# Autodesk Inventor assembly: 02하체
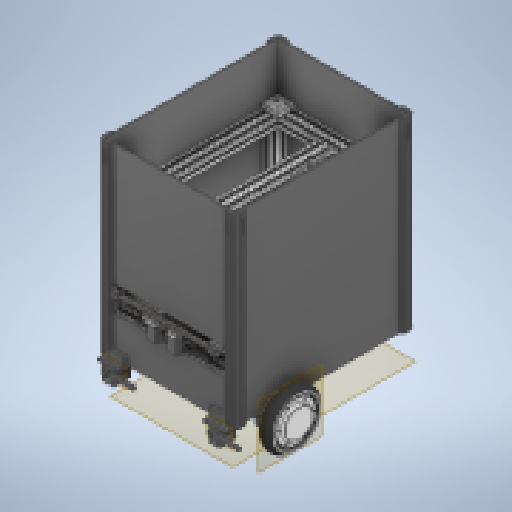
[picture p0: Inventor's stored thumbnail of the model, 512x512]
Saved by Autodesk Inventor 2026.2 (Build 302298010, 298A)
## iProperties
Created: 2026-03-27
Part Number: 02하체
Document SubType Name: Assembly
Designer: chanh
Author: chanh
## Documents named in this file (48)
- C:\Users\chanh\내 드라이브\교과공부\2026년 1학기 (4학년 1학기)\01창의제품설계\UMMA_CAD\02하체\02하체.iam
- C:\Users\chanh\내 드라이브\교과공부\2026년 1학기 (4학년 1학기)\01창의제품설계\UMMA_CAD\02하체\3060 Aluminium Profile 450mm.ipt
- C:\Users\chanh\내 드라이브\교과공부\2026년 1학기 (4학년 1학기)\01창의제품설계\UMMA_CAD\02하체\3060 Aluminium Profile 480mm.ipt
- C:\Users\chanh\내 드라이브\교과공부\2026년 1학기 (4학년 1학기)\01창의제품설계\UMMA_CAD\00부품\ZLLG80ASM250-L V3.0 (모터)\ZLLG80ASM250-L V3.0 Single shaft.iam
- C:\Users\chanh\내 드라이브\교과공부\2026년 1학기 (4학년 1학기)\01창의제품설계\UMMA_CAD\00부품\ZLAC8015D V4.0 (드라이버)\ZLAC8015D V4.0.iam
- C:\Users\chanh\내 드라이브\교과공부\2026년 1학기 (4학년 1학기)\01창의제품설계\UMMA_CAD\00부품\ZLLG80ASM250-L V3.0 (모터)\Nut.ipt
- C:\Users\chanh\내 드라이브\교과공부\2026년 1학기 (4학년 1학기)\01창의제품설계\UMMA_CAD\02하체\motor_bracket.ipt
- C:\Users\chanh\내 드라이브\교과공부\2026년 1학기 (4학년 1학기)\01창의제품설계\UMMA_CAD\02하체\Bottom_Plate_Acryl.ipt
- C:\Users\chanh\내 드라이브\교과공부\2026년 1학기 (4학년 1학기)\01창의제품설계\UMMA_CAD\02하체\Battery.ipt
- C:\Users\chanh\내 드라이브\교과공부\2026년 1학기 (4학년 1학기)\01창의제품설계\UMMA_CAD\02하체\assist_wheel.iam
- C:\Users\chanh\내 드라이브\교과공부\2026년 1학기 (4학년 1학기)\01창의제품설계\UMMA_CAD\02하체\assist_wheel_bracket.ipt
- C:\Users\chanh\내 드라이브\교과공부\2026년 1학기 (4학년 1학기)\01창의제품설계\UMMA_CAD\02하체\3060 Aluminium Profile 410mm.ipt
- C:\Users\chanh\내 드라이브\교과공부\2026년 1학기 (4학년 1학기)\01창의제품설계\UMMA_CAD\02하체\3060 Aluminium Profile 390mm.ipt
- C:\Users\chanh\내 드라이브\교과공부\2026년 1학기 (4학년 1학기)\01창의제품설계\UMMA_CAD\02하체\Linear Motor Bar (T-Frame).ipt
- C:\Users\chanh\내 드라이브\교과공부\2026년 1학기 (4학년 1학기)\01창의제품설계\UMMA_CAD\02하체\Linear Motor (T-Frame).ipt
- C:\Users\chanh\내 드라이브\교과공부\2026년 1학기 (4학년 1학기)\01창의제품설계\UMMA_CAD\02하체\Linear Motor Rear Braket.ipt
- C:\Users\chanh\내 드라이브\교과공부\2026년 1학기 (4학년 1학기)\01창의제품설계\UMMA_CAD\02하체\Linear Motor Front Braket.ipt
- C:\Users\chanh\내 드라이브\교과공부\2026년 1학기 (4학년 1학기)\01창의제품설계\UMMA_CAD\02하체\LMF20UU.ipt
- C:\Users\chanh\내 드라이브\교과공부\2026년 1학기 (4학년 1학기)\01창의제품설계\UMMA_CAD\02하체\Lift Bracket other side.ipt
- C:\Users\chanh\내 드라이브\교과공부\2026년 1학기 (4학년 1학기)\01창의제품설계\UMMA_CAD\02하체\Lift Bracket.ipt
- C:\Users\chanh\내 드라이브\교과공부\2026년 1학기 (4학년 1학기)\01창의제품설계\UMMA_CAD\02하체\MGN15C Cart.ipt
- C:\Users\chanh\내 드라이브\교과공부\2026년 1학기 (4학년 1학기)\01창의제품설계\UMMA_CAD\02하체\MGN15 Rail.ipt
- C:\Users\chanh\내 드라이브\교과공부\2026년 1학기 (4학년 1학기)\01창의제품설계\UMMA_CAD\02하체\Linear Motor Mount Right.ipt
- C:\Users\chanh\내 드라이브\교과공부\2026년 1학기 (4학년 1학기)\01창의제품설계\UMMA_CAD\02하체\Linear Motor Mount Left.ipt
- C:\Users\chanh\내 드라이브\교과공부\2026년 1학기 (4학년 1학기)\01창의제품설계\UMMA_CAD\02하체\LM Cart Braket.ipt
- C:\Users\chanh\내 드라이브\교과공부\2026년 1학기 (4학년 1학기)\01창의제품설계\UMMA_CAD\02하체\Space Craft Braket.ipt
- C:\Users\chanh\내 드라이브\교과공부\2026년 1학기 (4학년 1학기)\01창의제품설계\UMMA_CAD\02하체\LM20UU.ipt
- C:\Users\chanh\내 드라이브\교과공부\2026년 1학기 (4학년 1학기)\01창의제품설계\UMMA_CAD\02하체\Power Box (12V).ipt
- C:\Users\chanh\내 드라이브\교과공부\2026년 1학기 (4학년 1학기)\01창의제품설계\UMMA_CAD\02하체\Power Box (24V).ipt
- C:\Users\chanh\내 드라이브\교과공부\2026년 1학기 (4학년 1학기)\01창의제품설계\UMMA_CAD\02하체\Limit SW Bracket Right.ipt
- C:\Users\chanh\내 드라이브\교과공부\2026년 1학기 (4학년 1학기)\01창의제품설계\UMMA_CAD\02하체\Limit SW Bracket Left.ipt
- C:\Users\chanh\내 드라이브\교과공부\2026년 1학기 (4학년 1학기)\01창의제품설계\UMMA_CAD\02하체\RE38S-600Z-1M.ipt
- C:\Users\chanh\내 드라이브\교과공부\2026년 1학기 (4학년 1학기)\01창의제품설계\UMMA_CAD\02하체\Lift_encoder_frame.ipt
- C:\Users\chanh\내 드라이브\교과공부\2026년 1학기 (4학년 1학기)\01창의제품설계\UMMA_CAD\02하체\RE38S-600Z-1M-no-end.ipt
- C:\Users\chanh\내 드라이브\교과공부\2026년 1학기 (4학년 1학기)\01창의제품설계\UMMA_CAD\02하체\T-Frame_encoder_frame.ipt
- C:\Users\chanh\내 드라이브\교과공부\2026년 1학기 (4학년 1학기)\01창의제품설계\UMMA_CAD\02하체\LED Power Box (12V).ipt
- C:\Users\chanh\내 드라이브\교과공부\2026년 1학기 (4학년 1학기)\01창의제품설계\UMMA_CAD\02하체\LED Power Box (12V) Pillar.ipt
- C:\Users\chanh\내 드라이브\교과공부\2026년 1학기 (4학년 1학기)\01창의제품설계\UMMA_CAD\02하체\LED Power Box (12V) Cover.ipt
- C:\Users\chanh\내 드라이브\교과공부\2026년 1학기 (4학년 1학기)\01창의제품설계\UMMA_CAD\02하체\Power Box (24V) Cover.ipt
- C:\Users\chanh\내 드라이브\교과공부\2026년 1학기 (4학년 1학기)\01창의제품설계\UMMA_CAD\02하체\Power Box (12V) Cover.ipt
- C:\Users\chanh\내 드라이브\교과공부\2026년 1학기 (4학년 1학기)\01창의제품설계\UMMA_CAD\02하체\MGN15 Rail Middle.ipt
- C:\Users\chanh\내 드라이브\교과공부\2026년 1학기 (4학년 1학기)\01창의제품설계\UMMA_CAD\02하체\T-Frame Left Cover.ipt
- C:\Users\chanh\내 드라이브\교과공부\2026년 1학기 (4학년 1학기)\01창의제품설계\UMMA_CAD\02하체\T-Frame Right Cover.ipt
- C:\Users\chanh\내 드라이브\교과공부\2026년 1학기 (4학년 1학기)\01창의제품설계\UMMA_CAD\02하체\Foam Sheet Side.ipt
- C:\Users\chanh\내 드라이브\교과공부\2026년 1학기 (4학년 1학기)\01창의제품설계\UMMA_CAD\02하체\Foam Sheet Front.ipt
- C:\Users\chanh\내 드라이브\교과공부\2026년 1학기 (4학년 1학기)\01창의제품설계\UMMA_CAD\02하체\Foam Sheet Back.ipt
- C:\Users\chanh\내 드라이브\교과공부\2026년 1학기 (4학년 1학기)\01창의제품설계\UMMA_CAD\02하체\Foam Sheet Corner.ipt
- C:\Users\chanh\내 드라이브\교과공부\2026년 1학기 (4학년 1학기)\01창의제품설계\UMMA_CAD\02하체\Stopper\stopper.iam
## Components (79 placed, 47 different names)
1. stopper:1 [sub-assembly] — Mate:113, Flush:90, Mate:114
2. Lift Bracket:2 — Flush:59, Flush:60, Mate:40
3. Lift Bracket:1 — Flush:57, Mate:39, Flush:58
4. Lift Bracket other side:2 — Mate:42, Flush:63, Flush:64
5. Lift Bracket other side:1 — Mate:41, Flush:61, Flush:62
6. 3060 Aluminium Profile 480mm:1 — Mate:2, Flush:6, Flush:7, Mate:4, Flush:8, Flush:9, Flush:10, Flush:17, Mate:15, Mate:107, Flush:84
7. 3060 Aluminium Profile 480mm:2 — Mate:3, Flush:4, Flush:5, Flush:11, Mate:13, Mate:14, Mate:108, Flush:86
8. 3060 Aluminium Profile 480mm:3 — Flush:13, Mate:8, Flush:14, Mate:9
9. 3060 Aluminium Profile 480mm:4 — Flush:31, Mate:25, Flush:38
10. 3060 Aluminium Profile 480mm:5 — Flush:30, Mate:24, Flush:37
11. 3060 Aluminium Profile 480mm:6 — Flush:32, Mate:26, Flush:39, Flush:79, Mate:86, Mate:88, Flush:81
12. 3060 Aluminium Profile 480mm:7 — Mate:30, Flush:43, Flush:44, Mate:31, Flush:45, Mate:35, Flush:47, Mate:89, Mate:90, Mate:91, Mate:92, Mate:99
13. 3060 Aluminium Profile 450mm:1 — Flush:2, Mate:1, Flush:3, Mate:2, Mate:3, Flush:4, Flush:5, Flush:6, Flush:7, Mate:18, Mate:21, Flush:24, Flush:25, Flush:26, Flush:27, Flush:88, Flush:90, Mate:114
14. 3060 Aluminium Profile 450mm:2 — Mate:4, Flush:8, Flush:9, Flush:13, Mate:8, Mate:16, Flush:18, Mate:20, Flush:22, Flush:23, Mate:19, Flush:28, Flush:29, Mate:28
15. 3060 Aluminium Profile 450mm:3 — Mate:22, Flush:35, Flush:36, Mate:24, Flush:37, Mate:25, Flush:38, Mate:26, Flush:57, Mate:39, Flush:58, Mate:42, Flush:63, Flush:64, Mate:87
16. 3060 Aluminium Profile 450mm:4 — Mate:23, Flush:30, Flush:31, Flush:32, Flush:33, Flush:34, Flush:39, Flush:59, Flush:60, Mate:40, Mate:41, Flush:61, Flush:62
17. 3060 Aluminium Profile 410mm:1 — Mate:19, Flush:28, Flush:29, Mate:22, Mate:27, Flush:40
18. 3060 Aluminium Profile 410mm:2 — Mate:18, Flush:26, Flush:27, Mate:23, Mate:29, Flush:41, Mate:85, Flush:85
19. 3060 Aluminium Profile 410mm:3 — Mate:21, Flush:24, Flush:25, Flush:33, Flush:34, Mate:83, Flush:87
20. 3060 Aluminium Profile 410mm:4 — Mate:20, Flush:22, Flush:23, Flush:35, Flush:36
21. 3060 Aluminium Profile 390mm:1 — Mate:29, Flush:41, Flush:42, Flush:43, Flush:55, Mate:38, Flush:77, Mate:82, Mate:84, Flush:78, Mate:109
22. 3060 Aluminium Profile 390mm:2 — Mate:27, Flush:40, Mate:28, Flush:42, Mate:30, Flush:44, Flush:49, Flush:50, Mate:37, Mate:111
23. T-Frame Left Cover:1 — Rigid:21
24. T-Frame Right Cover:1 — Rigid:22
25. MGN15 Rail Middle:1 — Mate:106, Rotational:1
26. MGN15C Cart:4 — Rigid:20
27. MGN15C Cart:1 — Slider:2, Rigid:8
28. MGN15 Rail:1 — Slider:1, Slider:2, Rigid:21, Rigid:22, Rotational:1
29. MGN15C Cart:2 — Slider:1, Flush:67, Flush:68, Mate:67
30. Linear Motor Mount Right:1 — Rigid:7, Mate:72
31. Linear Motor Mount Left:1 — Rigid:9, Mate:73, Mate:105
32. LM Cart Braket:1 — Flush:67, Flush:68, Mate:67, Mate:72
33. LM Cart Braket:2 — Rigid:8, Mate:73, Mate:105
34. Space Craft Braket:1 — Rigid:10, Rigid:11, Mate:104, Rigid:20
35. LM20UU:1 — Rigid:10, Mate:69
36. LM20UU:2 — Rigid:11, Mate:68
37. Linear Motor Front Braket:1 — Flush:55, Flush:56, Mate:38, Rigid:5, Rigid:6, Mate:93, Mate:97, Angle:4, Mate:98, Angle:5
38. LMF20UU:1 — Rigid:5, Mate:104
39. LMF20UU:2 — Rigid:6
40. Linear Motor (T-Frame):1 — Mate:31, Flush:45, Mate:32, Angle:2, T자 왼쪽 거리, Flush:53
41. Linear Motor Bar (T-Frame):1 — Mate:32, Angle:2, T자 왼쪽 거리, Rigid:7, Mate:69
42. Linear Motor (T-Frame):2 — T자 오른쪽 거리, Mate:34, Angle:3, Mate:35, Flush:47, Flush:54
43. Linear Motor Bar (T-Frame):2 — T자 오른쪽 거리, Mate:34, Angle:3, Rigid:9, Mate:68
44. Linear Motor Rear Braket:1 — Flush:49, Flush:50, Mate:37, Flush:53, Flush:54, Mate:100, Mate:101
45. ZLLG80ASM250-L V3.0 Single shaft:1 [sub-assembly] — Rigid:3
46. ZLLG80ASM250-L V3.0 Single shaft:2 [sub-assembly] — Rigid:1
47. Nut:1 — Rigid:2
48. Nut:2 — Rigid:4
49. motor_bracket:1 — Flush:10, Flush:17, Rigid:1, Rigid:2, Mate:15
50. motor_bracket:2 — Flush:11, Mate:13, Rigid:3, Rigid:4, Mate:14
51. assist_wheel:1 [sub-assembly] — Tangent:1, Mate:17, Flush:20, Flush:21
52. assist_wheel_bracket:1 — Mate:16, Flush:18, Flush:19, Mate:17, Flush:20
53. Power Box (24V) Cover:1 — Rigid:18
54. Power Box (12V) Cover:1 — Rigid:19
55. ZLAC8015D V4.0:2 [sub-assembly] — Mate:102, Mate:103, Flush:83
56. LED Power Box (12V):1 — Rigid:15, Rigid:16, Rigid:17
57. LED Power Box (12V) Pillar:1 — Rigid:15
58. LED Power Box (12V) Pillar:2 — Rigid:16, Mate:99, Mate:100, Mate:101
59. LED Power Box (12V) Cover:1 — Rigid:17
60. Limit SW Bracket Right:1 — Flush:77, Mate:82, Mate:83
61. Limit SW Bracket Left:1 — Mate:84, Flush:78, Mate:85
62. Power Box (24V):1 — Mate:79, Mate:80, Mate:81, Rigid:18
63. Power Box (12V):1 — Mate:75, Flush:76, Mate:78, Mate:80, Rigid:19
64. Battery:1 — Mate:11, Flush:73, Flush:74, Mate:103, Flush:83
65. Bottom_Plate_Acryl:1 — Mate:9, Flush:15, Flush:16, Mate:11, Angle:1, Flush:74, Mate:75, Flush:76, Mate:79, Mate:102
66. RE38S-600Z-1M:1 — Flush:79, Mate:86, Mate:87, Flush:80
67. Lift_encoder_frame:1 — Flush:80, Mate:88, Flush:81
68. RE38S-600Z-1M-no-end:1 — Mate:92, Mate:89, Flush:82, Mate:93, Mate:94, Mate:95, Mate:96
69. RE38S-600Z-1M-no-end:2 — Mate:91, Mate:90, Flush:82, Rigid:14
70. T-Frame_encoder_frame:1 — Mate:94, Mate:95, Mate:96
71. T-Frame_encoder_frame:2 — Rigid:14
72. Foam Sheet Side:1 — Mate:107, Flush:84, Flush:85, Flush:89, Mate:112, Rigid:24
73. Foam Sheet Side:2 — Mate:108, Flush:86, Flush:87, Mate:110, Rigid:23, Rigid:26
74. Foam Sheet Front:1 — Mate:109, Flush:88, Mate:110, Mate:113
75. Foam Sheet Back:1 — Mate:111, Flush:89, Mate:112, Rigid:25
76. Foam Sheet Corner:1 — Rigid:23
77. Foam Sheet Corner:2 — Rigid:25
78. Foam Sheet Corner:3 — Rigid:26
79. Foam Sheet Corner:4 — Rigid:24
## Relationships (191: Mate 80, Flush 78, WeldJoint 24, Angle 5, TranslationJoint 2, Tangent 1, RevoluteJoint 1)
- T자 왼쪽 거리 [Mate] (87 mm): Linear Motor (T-Frame):1 ↔ Linear Motor Bar (T-Frame):1
- T자 오른쪽 거리 [Mate] (87 mm): Linear Motor (T-Frame):2 ↔ Linear Motor Bar (T-Frame):2
- Flush:1 (-240 mm)
- Flush:2: 3060 Aluminium Profile 450mm:1
- Mate:1: 3060 Aluminium Profile 450mm:1
- Flush:3: 3060 Aluminium Profile 450mm:1
- Mate:2: 3060 Aluminium Profile 480mm:1 ↔ 3060 Aluminium Profile 450mm:1
- Mate:3: 3060 Aluminium Profile 480mm:2 ↔ 3060 Aluminium Profile 450mm:1
- Flush:4: 3060 Aluminium Profile 480mm:2 ↔ 3060 Aluminium Profile 450mm:1
- Flush:5: 3060 Aluminium Profile 480mm:2 ↔ 3060 Aluminium Profile 450mm:1
- Flush:6: 3060 Aluminium Profile 480mm:1 ↔ 3060 Aluminium Profile 450mm:1
- Flush:7: 3060 Aluminium Profile 480mm:1 ↔ 3060 Aluminium Profile 450mm:1
- Mate:4: 3060 Aluminium Profile 480mm:1 ↔ 3060 Aluminium Profile 450mm:2
- Flush:8: 3060 Aluminium Profile 480mm:1 ↔ 3060 Aluminium Profile 450mm:2
- Flush:9: 3060 Aluminium Profile 480mm:1 ↔ 3060 Aluminium Profile 450mm:2
- Flush:10: 3060 Aluminium Profile 480mm:1 ↔ motor_bracket:1
- Flush:17 (150 mm): 3060 Aluminium Profile 480mm:1 ↔ motor_bracket:1
- Rigid:1 [WeldJoint]: ZLLG80ASM250-L V3.0 Single shaft:2 ↔ motor_bracket:1
- Rigid:2 [WeldJoint]: Nut:1 ↔ motor_bracket:1
- Flush:11: 3060 Aluminium Profile 480mm:2 ↔ motor_bracket:2
- Mate:13 (-150 mm): 3060 Aluminium Profile 480mm:2 ↔ motor_bracket:2
- Rigid:3 [WeldJoint]: ZLLG80ASM250-L V3.0 Single shaft:1 ↔ motor_bracket:2
- Rigid:4 [WeldJoint]: Nut:2 ↔ motor_bracket:2
- Flush:13: 3060 Aluminium Profile 480mm:3 ↔ 3060 Aluminium Profile 450mm:2
- Mate:8: 3060 Aluminium Profile 480mm:3 ↔ 3060 Aluminium Profile 450mm:2
- Flush:14: 3060 Aluminium Profile 480mm:3
- Mate:9: 3060 Aluminium Profile 480mm:3 ↔ Bottom_Plate_Acryl:1
- Flush:15: Bottom_Plate_Acryl:1
- Flush:16: Bottom_Plate_Acryl:1
- Mate:11: Battery:1 ↔ Bottom_Plate_Acryl:1
- Mate:14: 3060 Aluminium Profile 480mm:2 ↔ motor_bracket:2
- Mate:15: 3060 Aluminium Profile 480mm:1 ↔ motor_bracket:1
- Angle:1 (0 deg): Bottom_Plate_Acryl:1
- Tangent:1: assist_wheel:1
- Mate:16: 3060 Aluminium Profile 450mm:2 ↔ assist_wheel_bracket:1
- Flush:18: 3060 Aluminium Profile 450mm:2 ↔ assist_wheel_bracket:1
- Flush:19: assist_wheel_bracket:1
- Mate:17: assist_wheel:1 ↔ assist_wheel_bracket:1
- Flush:20: assist_wheel:1 ↔ assist_wheel_bracket:1
- Flush:21: assist_wheel:1
- Mate:18: 3060 Aluminium Profile 450mm:1 ↔ 3060 Aluminium Profile 410mm:2
- Mate:19: 3060 Aluminium Profile 450mm:2 ↔ 3060 Aluminium Profile 410mm:1
- Mate:20: 3060 Aluminium Profile 450mm:2 ↔ 3060 Aluminium Profile 410mm:4
- Mate:21: 3060 Aluminium Profile 450mm:1 ↔ 3060 Aluminium Profile 410mm:3
- Flush:22: 3060 Aluminium Profile 450mm:2 ↔ 3060 Aluminium Profile 410mm:4
- Flush:23: 3060 Aluminium Profile 450mm:2 ↔ 3060 Aluminium Profile 410mm:4
- Flush:24: 3060 Aluminium Profile 450mm:1 ↔ 3060 Aluminium Profile 410mm:3
- Flush:25: 3060 Aluminium Profile 450mm:1 ↔ 3060 Aluminium Profile 410mm:3
- Flush:26: 3060 Aluminium Profile 450mm:1 ↔ 3060 Aluminium Profile 410mm:2
- Flush:27: 3060 Aluminium Profile 450mm:1 ↔ 3060 Aluminium Profile 410mm:2
- Flush:28: 3060 Aluminium Profile 450mm:2 ↔ 3060 Aluminium Profile 410mm:1
- Flush:29: 3060 Aluminium Profile 450mm:2 ↔ 3060 Aluminium Profile 410mm:1
- Mate:22: 3060 Aluminium Profile 450mm:3 ↔ 3060 Aluminium Profile 410mm:1
- Mate:23: 3060 Aluminium Profile 450mm:4 ↔ 3060 Aluminium Profile 410mm:2
- Flush:30: 3060 Aluminium Profile 480mm:5 ↔ 3060 Aluminium Profile 450mm:4
- Flush:31: 3060 Aluminium Profile 480mm:4 ↔ 3060 Aluminium Profile 450mm:4
- Flush:32: 3060 Aluminium Profile 480mm:6 ↔ 3060 Aluminium Profile 450mm:4
- Flush:33: 3060 Aluminium Profile 450mm:4 ↔ 3060 Aluminium Profile 410mm:3
- Flush:34: 3060 Aluminium Profile 450mm:4 ↔ 3060 Aluminium Profile 410mm:3
- Flush:35: 3060 Aluminium Profile 450mm:3 ↔ 3060 Aluminium Profile 410mm:4
- Flush:36: 3060 Aluminium Profile 450mm:3 ↔ 3060 Aluminium Profile 410mm:4
- Mate:24: 3060 Aluminium Profile 480mm:5 ↔ 3060 Aluminium Profile 450mm:3
- Flush:37: 3060 Aluminium Profile 480mm:5 ↔ 3060 Aluminium Profile 450mm:3
- Mate:25: 3060 Aluminium Profile 480mm:4 ↔ 3060 Aluminium Profile 450mm:3
- Flush:38: 3060 Aluminium Profile 480mm:4 ↔ 3060 Aluminium Profile 450mm:3
- Mate:26: 3060 Aluminium Profile 480mm:6 ↔ 3060 Aluminium Profile 450mm:3
- Flush:39: 3060 Aluminium Profile 480mm:6 ↔ 3060 Aluminium Profile 450mm:4
- Mate:27: 3060 Aluminium Profile 410mm:1 ↔ 3060 Aluminium Profile 390mm:2
- Flush:40: 3060 Aluminium Profile 410mm:1 ↔ 3060 Aluminium Profile 390mm:2
- Mate:28 (80 mm): 3060 Aluminium Profile 450mm:2 ↔ 3060 Aluminium Profile 390mm:2
- Mate:29: 3060 Aluminium Profile 410mm:2 ↔ 3060 Aluminium Profile 390mm:1
- Flush:41: 3060 Aluminium Profile 410mm:2 ↔ 3060 Aluminium Profile 390mm:1
- Flush:42: 3060 Aluminium Profile 390mm:1 ↔ 3060 Aluminium Profile 390mm:2
- Mate:30: 3060 Aluminium Profile 480mm:7 ↔ 3060 Aluminium Profile 390mm:2
- Flush:43: 3060 Aluminium Profile 480mm:7 ↔ 3060 Aluminium Profile 390mm:1
- Flush:44: 3060 Aluminium Profile 480mm:7 ↔ 3060 Aluminium Profile 390mm:2
- Mate:31 (10 mm): 3060 Aluminium Profile 480mm:7 ↔ Linear Motor (T-Frame):1
- Flush:45 (-35 mm): 3060 Aluminium Profile 480mm:7 ↔ Linear Motor (T-Frame):1
- Mate:32: Linear Motor (T-Frame):1 ↔ Linear Motor Bar (T-Frame):1
- Angle:2 (-20 deg): Linear Motor (T-Frame):1 ↔ Linear Motor Bar (T-Frame):1
- Mate:34: Linear Motor (T-Frame):2 ↔ Linear Motor Bar (T-Frame):2
- Angle:3 (20 deg): Linear Motor (T-Frame):2 ↔ Linear Motor Bar (T-Frame):2
- Mate:35 (10 mm): 3060 Aluminium Profile 480mm:7 ↔ Linear Motor (T-Frame):2
- Flush:47 (-35 mm): 3060 Aluminium Profile 480mm:7 ↔ Linear Motor (T-Frame):2
- Flush:49: 3060 Aluminium Profile 390mm:2 ↔ Linear Motor Rear Braket:1
- Flush:50: 3060 Aluminium Profile 390mm:2 ↔ Linear Motor Rear Braket:1
- Mate:37: 3060 Aluminium Profile 390mm:2 ↔ Linear Motor Rear Braket:1
- Flush:53 (15 mm): Linear Motor (T-Frame):1 ↔ Linear Motor Rear Braket:1
- Flush:54 (15 mm): Linear Motor (T-Frame):2 ↔ Linear Motor Rear Braket:1
- Flush:55 (60 mm): 3060 Aluminium Profile 390mm:1 ↔ Linear Motor Front Braket:1
- Flush:56: Linear Motor Front Braket:1
- Mate:38: 3060 Aluminium Profile 390mm:1 ↔ Linear Motor Front Braket:1
- Rigid:5 [WeldJoint]: Linear Motor Front Braket:1 ↔ LMF20UU:1
- Rigid:6 [WeldJoint]: Linear Motor Front Braket:1 ↔ LMF20UU:2
- Flush:57: Lift Bracket:1 ↔ 3060 Aluminium Profile 450mm:3
- Mate:39: Lift Bracket:1 ↔ 3060 Aluminium Profile 450mm:3
- Flush:58 (1 mm): Lift Bracket:1 ↔ 3060 Aluminium Profile 450mm:3
- Flush:59: Lift Bracket:2 ↔ 3060 Aluminium Profile 450mm:4
- Flush:60 (1 mm): Lift Bracket:2 ↔ 3060 Aluminium Profile 450mm:4
- Mate:40: Lift Bracket:2 ↔ 3060 Aluminium Profile 450mm:4
- Mate:41: Lift Bracket other side:1 ↔ 3060 Aluminium Profile 450mm:4
- Flush:61 (1 mm): Lift Bracket other side:1 ↔ 3060 Aluminium Profile 450mm:4
- Flush:62: Lift Bracket other side:1 ↔ 3060 Aluminium Profile 450mm:4
- Mate:42: Lift Bracket other side:2 ↔ 3060 Aluminium Profile 450mm:3
- Flush:63: Lift Bracket other side:2 ↔ 3060 Aluminium Profile 450mm:3
- Flush:64 (1 mm): Lift Bracket other side:2 ↔ 3060 Aluminium Profile 450mm:3
- Slider:1 [TranslationJoint]: MGN15 Rail:1 ↔ MGN15C Cart:2
- Slider:2 [TranslationJoint]: MGN15C Cart:1 ↔ MGN15 Rail:1
- Rigid:7 [WeldJoint]: Linear Motor Mount Right:1 ↔ Linear Motor Bar (T-Frame):1
- Flush:67: MGN15C Cart:2 ↔ LM Cart Braket:1
- Flush:68: MGN15C Cart:2 ↔ LM Cart Braket:1
- Mate:67: MGN15C Cart:2 ↔ LM Cart Braket:1
- Rigid:8 [WeldJoint]: MGN15C Cart:1 ↔ LM Cart Braket:2
- Rigid:9 [WeldJoint]: Linear Motor Mount Left:1 ↔ Linear Motor Bar (T-Frame):2
- Rigid:10 [WeldJoint]: Space Craft Braket:1 ↔ LM20UU:1
- Rigid:11 [WeldJoint]: Space Craft Braket:1 ↔ LM20UU:2
- Mate:68: LM20UU:2 ↔ Linear Motor Bar (T-Frame):2
- Mate:69: LM20UU:1 ↔ Linear Motor Bar (T-Frame):1
- Mate:72: Linear Motor Mount Right:1 ↔ LM Cart Braket:1
- Mate:73: Linear Motor Mount Left:1 ↔ LM Cart Braket:2
- Flush:73: Battery:1
- Flush:74: Battery:1 ↔ Bottom_Plate_Acryl:1
- Mate:75: Power Box (12V):1 ↔ Bottom_Plate_Acryl:1
- Flush:76: Power Box (12V):1 ↔ Bottom_Plate_Acryl:1
- Mate:78: Power Box (12V):1
- Mate:79: Power Box (24V):1 ↔ Bottom_Plate_Acryl:1
- Mate:80 (15 mm): Power Box (24V):1 ↔ Power Box (12V):1
- Mate:81: Power Box (24V):1
- Flush:77: 3060 Aluminium Profile 390mm:1 ↔ Limit SW Bracket Right:1
- Mate:82: 3060 Aluminium Profile 390mm:1 ↔ Limit SW Bracket Right:1
- Mate:83 (70 mm): 3060 Aluminium Profile 410mm:3 ↔ Limit SW Bracket Right:1
- Mate:84: 3060 Aluminium Profile 390mm:1 ↔ Limit SW Bracket Left:1
- Flush:78: 3060 Aluminium Profile 390mm:1 ↔ Limit SW Bracket Left:1
- Mate:85 (70 mm): 3060 Aluminium Profile 410mm:2 ↔ Limit SW Bracket Left:1
- Flush:79: 3060 Aluminium Profile 480mm:6 ↔ RE38S-600Z-1M:1
- Mate:86: 3060 Aluminium Profile 480mm:6 ↔ RE38S-600Z-1M:1
- Mate:87 (70 mm): 3060 Aluminium Profile 450mm:3 ↔ RE38S-600Z-1M:1
- Flush:80: RE38S-600Z-1M:1 ↔ Lift_encoder_frame:1
- Mate:88: 3060 Aluminium Profile 480mm:6 ↔ Lift_encoder_frame:1
- Flush:81: 3060 Aluminium Profile 480mm:6 ↔ Lift_encoder_frame:1
- Mate:91 (4 mm): 3060 Aluminium Profile 480mm:7 ↔ RE38S-600Z-1M-no-end:2
- Mate:92 (4 mm): 3060 Aluminium Profile 480mm:7 ↔ RE38S-600Z-1M-no-end:1
- Mate:89 (20 mm): 3060 Aluminium Profile 480mm:7 ↔ RE38S-600Z-1M-no-end:1
- Mate:90 (20 mm): 3060 Aluminium Profile 480mm:7 ↔ RE38S-600Z-1M-no-end:2
- Flush:82: RE38S-600Z-1M-no-end:1 ↔ RE38S-600Z-1M-no-end:2
- Mate:93 (30 mm): Linear Motor Front Braket:1 ↔ RE38S-600Z-1M-no-end:1
- Mate:94: RE38S-600Z-1M-no-end:1 ↔ T-Frame_encoder_frame:1
- Mate:95: RE38S-600Z-1M-no-end:1 ↔ T-Frame_encoder_frame:1
- Mate:96: RE38S-600Z-1M-no-end:1 ↔ T-Frame_encoder_frame:1
- Rigid:14 [WeldJoint]: RE38S-600Z-1M-no-end:2 ↔ T-Frame_encoder_frame:2
- Mate:97: Linear Motor Front Braket:1
- Angle:4 (0 deg): Linear Motor Front Braket:1
- Mate:98: Linear Motor Front Braket:1
- Angle:5 (0 deg): Linear Motor Front Braket:1
- Rigid:15 [WeldJoint]: LED Power Box (12V):1 ↔ LED Power Box (12V) Pillar:1
- Rigid:16 [WeldJoint]: LED Power Box (12V):1 ↔ LED Power Box (12V) Pillar:2
- Mate:99: 3060 Aluminium Profile 480mm:7 ↔ LED Power Box (12V) Pillar:2
- Mate:100 (10 mm): Linear Motor Rear Braket:1 ↔ LED Power Box (12V) Pillar:2
- Mate:101: Linear Motor Rear Braket:1 ↔ LED Power Box (12V) Pillar:2
- Rigid:17 [WeldJoint]: LED Power Box (12V):1 ↔ LED Power Box (12V) Cover:1
- Rigid:18 [WeldJoint]: Power Box (24V) Cover:1 ↔ Power Box (24V):1
- Mate:102: ZLAC8015D V4.0:2 ↔ Bottom_Plate_Acryl:1
- Mate:103: ZLAC8015D V4.0:2 ↔ Battery:1
- Flush:83: ZLAC8015D V4.0:2 ↔ Battery:1
- Rigid:19 [WeldJoint]: Power Box (12V) Cover:1 ↔ Power Box (12V):1
- Mate:104: Space Craft Braket:1 ↔ LMF20UU:1
- Rigid:20 [WeldJoint]: MGN15C Cart:4 ↔ Space Craft Braket:1
- Mate:105: Linear Motor Mount Left:1 ↔ LM Cart Braket:2
- Mate:106: MGN15 Rail Middle:1
- Rigid:21 [WeldJoint]: T-Frame Left Cover:1 ↔ MGN15 Rail:1
- Rigid:22 [WeldJoint]: T-Frame Right Cover:1 ↔ MGN15 Rail:1
- Rotational:1 [RevoluteJoint]: MGN15 Rail Middle:1 ↔ MGN15 Rail:1
- Mate:107: 3060 Aluminium Profile 480mm:1 ↔ Foam Sheet Side:1
- Flush:84: 3060 Aluminium Profile 480mm:1 ↔ Foam Sheet Side:1
- Flush:85: 3060 Aluminium Profile 410mm:2 ↔ Foam Sheet Side:1
- Mate:108: 3060 Aluminium Profile 480mm:2 ↔ Foam Sheet Side:2
- Flush:86: 3060 Aluminium Profile 480mm:2 ↔ Foam Sheet Side:2
- Flush:87: 3060 Aluminium Profile 410mm:3 ↔ Foam Sheet Side:2
- Mate:109: 3060 Aluminium Profile 390mm:1 ↔ Foam Sheet Front:1
- Flush:88: 3060 Aluminium Profile 450mm:1 ↔ Foam Sheet Front:1
- Mate:110: Foam Sheet Side:2 ↔ Foam Sheet Front:1
- Mate:111: 3060 Aluminium Profile 390mm:2 ↔ Foam Sheet Back:1
- Flush:89: Foam Sheet Side:1 ↔ Foam Sheet Back:1
- Mate:112: Foam Sheet Side:1 ↔ Foam Sheet Back:1
- Rigid:23 [WeldJoint]: Foam Sheet Side:2 ↔ Foam Sheet Corner:1
- Rigid:24 [WeldJoint]: Foam Sheet Side:1 ↔ Foam Sheet Corner:4
- Rigid:25 [WeldJoint]: Foam Sheet Back:1 ↔ Foam Sheet Corner:2
- Rigid:26 [WeldJoint]: Foam Sheet Side:2 ↔ Foam Sheet Corner:3
- Mate:113: stopper:1 ↔ Foam Sheet Front:1
- Flush:90: stopper:1 ↔ 3060 Aluminium Profile 450mm:1
- Mate:114: stopper:1 ↔ 3060 Aluminium Profile 450mm:1
